# Autodesk Inventor assembly: 71. Блок шестерен заднего хода
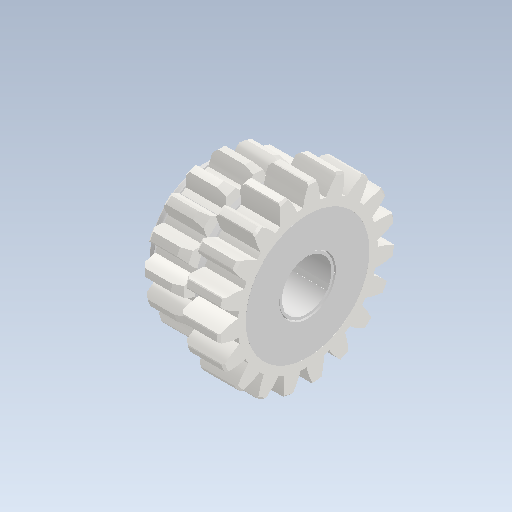
[picture p0: Inventor's stored thumbnail of the model, 512x512]
Saved by Autodesk Inventor 2021 (Build 250183000, 183)
## iProperties
Created: 2021-03-24
Part Number: 71. Блок шестерен заднего хода
Document SubType Name: Assembly
Designer: Данил
Author: Данил
## Documents named in this file (5)
- C:\Users\Данил\Desktop\Коробка передач\Детали\71. Блок шестерен заднего хода.iam
- C:\Users\Данил\Desktop\Коробка передач\Детали\71. Блок шестерен заднего хода.ipt
- C:\Users\Данил\Desktop\Коробка передач\Детали\71. Блок шестерен заднего хода\Мастер проектирования\Цилиндрическое зубчатое зацепление1.iam
- C:\Users\Данил\Desktop\Коробка передач\Детали\71. Блок шестерен заднего хода\Мастер проектирования\Цилиндрическое зубчатое зацепление2.iam
- C:\Users\Данил\Desktop\Коробка передач\Детали\71. Втулка блока заднего хода.ipt
## Components (4 placed, 3 different names)
1. 71. Блок шестерен заднего хода:1 — Совмещение:1, Заподлицо:1, Совмещение:2, Совмещение:3, Совмещение:4, Заподлицо:2
2. Цилиндрическое зубчатое зацепление:1 [sub-assembly] — Совмещение:1, Заподлицо:1
3. Цилиндрическое зубчатое зацепление:2 [sub-assembly] — Совмещение:2, Совмещение:3
4. 71. Втулка блока заднего хода:1 — Совмещение:4, Заподлицо:2
## Relationships (6: Mate 4, Flush 2)
- Совмещение:1 [Mate]: 71. Блок шестерен заднего хода:1 ↔ Цилиндрическое зубчатое зацепление:1
- Заподлицо:1 [Flush]: 71. Блок шестерен заднего хода:1 ↔ Цилиндрическое зубчатое зацепление:1
- Совмещение:2 [Mate]: 71. Блок шестерен заднего хода:1 ↔ Цилиндрическое зубчатое зацепление:2
- Совмещение:3 [Mate]: 71. Блок шестерен заднего хода:1 ↔ Цилиндрическое зубчатое зацепление:2
- Совмещение:4 [Mate]: 71. Блок шестерен заднего хода:1 ↔ 71. Втулка блока заднего хода:1
- Заподлицо:2 [Flush] (0.5 mm): 71. Блок шестерен заднего хода:1 ↔ 71. Втулка блока заднего хода:1
